# Autodesk Inventor assembly: 0306_MotorMountMain_qty4
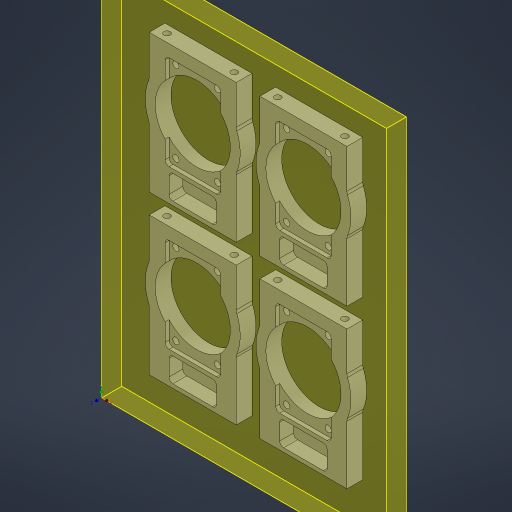
[picture p0: Inventor's stored thumbnail of the model, 512x512]
Saved by Autodesk Inventor 2024.2 (Build 282272000, 272)
## iProperties
Created: 2024-03-05
Part Number: 0306_MotorMountMain_qty4
Document SubType Name: Assembly
Designer: Hanaoka
Author: Hanaoka
## Documents named in this file (2)
- G:\共有ドライブ\reRo\05_個人\hanaoka\inventor\CAMpath\0306_MotorMountMain_qty4.iam
- G:\共有ドライブ\reRo\05_個人\hanaoka\inventor\DriveUnit\MotorMount_main.ipt
## Components (4 placed, 1 different names)
1. MotorMount_main:1 — メイト:1, メイト:2, 正接:1
2. MotorMount_main:2
3. MotorMount_main:3
4. MotorMount_main:4
## Component patterns: (4 elements, first: MotorMount_main:1)
## Relationships (3: Mate 2, Tangent 1)
- メイト:1 [Mate]: MotorMount_main:1
- メイト:2 [Mate]: MotorMount_main:1
- 正接:1 [Tangent]: MotorMount_main:1
